# Autodesk Inventor assembly: Assembly_Cube_empty_1x1_v2
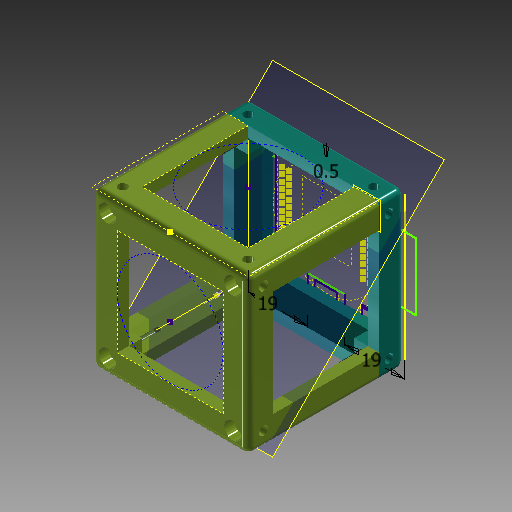
[picture p0: Inventor's stored thumbnail of the model, 512x512]
Saved by Autodesk Inventor 2019.4 (Build 234330000, 330)
## iProperties
Created: 2018-06-11
Part Number: Assembly_Cube_empty_1x1_v2
Material: Generisch
Document SubType Name: Assembly
Designer: diederichbenedict
Mass: 28.3962 g
Surface Area: 161.576 cm^2
Volume: 24.38 cm^3
Density: 1.16473 g/cm^3
Author: diederichbenedict
## Documents named in this file (4)
- D:\Dropbox\UC2\02_CAD\INVENTOR\uc2_v2\Assembly_Cube_empty_1x1_v2.iam
- D:\Dropbox\UC2\02_CAD\INVENTOR\uc2_v2\10_Cube_1x1_v2.ipt
- D:\Dropbox\UC2\02_CAD\INVENTOR\uc2_v2\10_Lid_1x1_v2.ipt
- D:\Dropbox\UC2\02_CAD\INVENTOR\uc2_v2\DIN 912 - M3 x 0,5 x 12 x 10,75.ipt
## Components (6 placed, 3 different names)
1. 10_Cube_1x1_v2:1 — Mate:3, Mate:2
2. 10_Lid_1x1_v2:1 — Mate:3, Mate:2, Flush:3, Flush:4, Flush:5, Insert:20, Insert:21, Insert:22, Insert:23
3. DIN 912 - ersetzt durch DIN EN ISO 4762 M3 x 12:5 — Insert:21
4. DIN 912 - ersetzt durch DIN EN ISO 4762 M3 x 12:6 — Insert:23
5. DIN 912 - ersetzt durch DIN EN ISO 4762 M3 x 12:7 — Insert:20
6. DIN 912 - ersetzt durch DIN EN ISO 4762 M3 x 12:8 — Insert:22
## Relationships (9: Insert 4, Flush 3, Mate 2)
- Mate:3: 10_Cube_1x1_v2:1 ↔ 10_Lid_1x1_v2:1
- Mate:2: 10_Cube_1x1_v2:1 ↔ 10_Lid_1x1_v2:1
- Flush:3: 10_Lid_1x1_v2:1
- Flush:4: 10_Lid_1x1_v2:1
- Flush:5: 10_Lid_1x1_v2:1
- Insert:20: 10_Lid_1x1_v2:1 ↔ DIN 912 - ersetzt durch DIN EN ISO 4762 M3 x 12:7
- Insert:21: 10_Lid_1x1_v2:1 ↔ DIN 912 - ersetzt durch DIN EN ISO 4762 M3 x 12:5
- Insert:22: 10_Lid_1x1_v2:1 ↔ DIN 912 - ersetzt durch DIN EN ISO 4762 M3 x 12:8
- Insert:23: 10_Lid_1x1_v2:1 ↔ DIN 912 - ersetzt durch DIN EN ISO 4762 M3 x 12:6
